# Autodesk Inventor assembly: Colossus_7kW
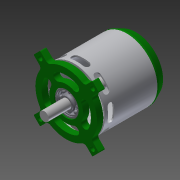
[picture p0: Inventor's stored thumbnail of the model, 180x180]
Saved by Autodesk Inventor 2014 (Build 180170000, 170)
## iProperties
Created: 2014-11-23
Part Number: Colossus_7kW
Document SubType Name: Assembly
Designer: Yann
Author: Yann
## Documents named in this file (6)
- C:\Users\Yann\Documents\GitHub\Velocar_CAD\Workspaces\Espace de travail\Source\Rear_train\Motor_Outrunner\Colossus_7kW.iam
- C:\Users\Yann\Documents\GitHub\Velocar_CAD\Workspaces\Espace de travail\Source\Rear_train\Motor_Outrunner\Colossus_7kW_Stator.ipt
- C:\Users\Yann\Documents\GitHub\Velocar_CAD\Workspaces\Espace de travail\Source\Rear_train\Motor_Outrunner\Colossus_7kW_Rotor.ipt
- C:\Users\Yann\Documents\GitHub\Velocar_CAD\Workspaces\Espace de travail\Source\Rear_train\Motor_Outrunner\Colossus_7kW_Rotor_body.ipt
- C:\Users\Yann\Documents\GitHub\Velocar_CAD\Workspaces\Espace de travail\Source\Rear_train\Motor_Outrunner\Colossus_7kW_Shaft.ipt
- C:\Users\Yann\Documents\GitHub\Velocar_CAD\Libraries\Content Center Files\fr-FR\ANSI AFBMA 16.1(0)\ANSI_AFBMA 16.1 - 12 x 32 x 16.ipt
## Components (6 placed, 5 different names)
1. Colossus_7kW_Stator:1 — Affleurement:1, Affleurement:2, Affleurement:3, Rotation:1
2. Colossus_7kW_Rotor:1 — Affleurement:4, Affleurement:5, Affleurement:6, Placage:1, Placage:2, Rotation:2
3. Colossus_7kW_Rotor_body:1 — Affleurement:7, Affleurement:8, Placage:1
4. Colossus_7kW_Shaft:1 — Affleurement:9, Affleurement:10, Placage:2
5. ANSI/AFBMA 16.1 - Roulements à billes aéro: deux rangées, fixe, diamètre de série 2 12 x 32 x 16:1 — Rotation:2
6. ANSI/AFBMA 16.1 - Roulements à billes aéro: deux rangées, fixe, diamètre de série 2 12 x 32 x 16:2 — Rotation:1
## Relationships (14: Flush 10, Mate 2, RevoluteJoint 2)
- Affleurement:1 [Flush]: Colossus_7kW_Stator:1
- Affleurement:2 [Flush]: Colossus_7kW_Stator:1
- Affleurement:3 [Flush]: Colossus_7kW_Stator:1
- Affleurement:4 [Flush]: Colossus_7kW_Rotor:1
- Affleurement:5 [Flush]: Colossus_7kW_Rotor:1
- Affleurement:6 [Flush] (90.322 mm): Colossus_7kW_Rotor:1
- Affleurement:7 [Flush]: Colossus_7kW_Rotor_body:1
- Affleurement:8 [Flush]: Colossus_7kW_Rotor_body:1
- Placage:1 [Mate]: Colossus_7kW_Rotor:1 ↔ Colossus_7kW_Rotor_body:1
- Affleurement:9 [Flush]: Colossus_7kW_Shaft:1
- Affleurement:10 [Flush]: Colossus_7kW_Shaft:1
- Placage:2 [Mate]: Colossus_7kW_Rotor:1 ↔ Colossus_7kW_Shaft:1
- Rotation:1 [RevoluteJoint]: Colossus_7kW_Stator:1 ↔ ANSI/AFBMA 16.1 - Roulements à billes aéro: deux rangées, fixe, diamètre de série 2 12 x 32 x 16:2
- Rotation:2 [RevoluteJoint]: Colossus_7kW_Rotor:1 ↔ ANSI/AFBMA 16.1 - Roulements à billes aéro: deux rangées, fixe, diamètre de série 2 12 x 32 x 16:1
